# Autodesk Inventor assembly: s-assy-link2+3+4+5+gripper
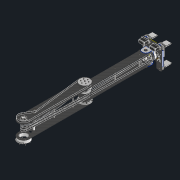
[picture p0: Inventor's stored thumbnail of the model, 180x180]
Saved by Autodesk Inventor 2021 (Build 250183000, 183)
## iProperties
Created: 2021-08-13
Part Number: s-assy-link2+3+4+5+gripper
Document SubType Name: Assembly
Designer: yuta0
Author: yuta0
## Documents named in this file (3)
- C:\Users\yuta0\Documents\GitHub\catchrobo_hardware\assy-robot\s-assy-link2+3+4+5+gripper.iam
- C:\Users\yuta0\Documents\GitHub\catchrobo_hardware\assy-robot\s-assy-link2.iam
- C:\Users\yuta0\Documents\GitHub\catchrobo_hardware\assy-robot\s-assy-link3+4+5+gripper.iam
## Components (2 placed, 2 different names)
1. s-assy-link2:1 [sub-assembly] — メイト:1, メイト:2
2. s-assy-link3+4+5+gripper:1 [sub-assembly] — メイト:1, メイト:2, 角度:2
## Relationships (3: Mate 2, Angle 1)
- メイト:1 [Mate]: s-assy-link2:1 ↔ s-assy-link3+4+5+gripper:1
- メイト:2 [Mate]: s-assy-link2:1 ↔ s-assy-link3+4+5+gripper:1
- 角度:2 [Angle] (0 deg): s-assy-link3+4+5+gripper:1
